# Autodesk Inventor assembly: WristDifferential
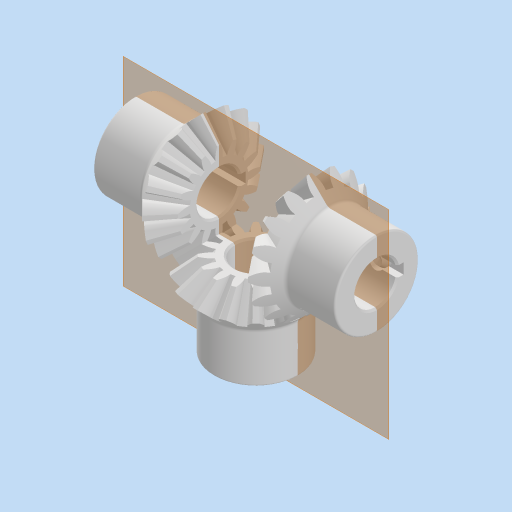
[picture p0: Inventor's stored thumbnail of the model, 512x512]
Saved by Autodesk Inventor 2024 (Build 280153000, 153)
## iProperties
Created: 2023-11-15
Part Number: WristDifferential
Document SubType Name: Assembly
Designer: megan
Author: megan
## Documents named in this file (2)
- C:\Users\megan\OneDrive\Documents\GitHub\BehrendURCMechanical\CAD\Chassis V3\Wrist\WristDifferential.iam
- C:\Users\megan\Downloads\6843K11_Metal Miter Gear\6843K11_Metal Miter Gear.ipt
## Components (3 placed, 1 different names)
1. 6843K11_Metal Miter Gear:1 — Mate:3
2. 6843K11_Metal Miter Gear:2 — Mate:1, Mate:2
3. 6843K11_Metal Miter Gear:3 — Mate:1
## Relationships (3: Mate 3)
- Mate:1: 6843K11_Metal Miter Gear:2 ↔ 6843K11_Metal Miter Gear:3
- Mate:2: 6843K11_Metal Miter Gear:2
- Mate:3: 6843K11_Metal Miter Gear:1
